# Autodesk Inventor assembly: Rail_assy
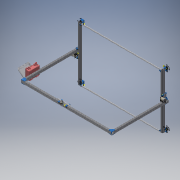
[picture p0: Inventor's stored thumbnail of the model, 180x180]
Saved by Autodesk Inventor 2019.4 (Build 234330000, 330)
## iProperties
Created: 2021-02-01
Part Number: Rail_assy
Document SubType Name: Assembly
Designer: Jorian Brusind
Author: Jorian Brusind
## Documents named in this file (12)
- C:\Users\Jorian Brusind\Documents\GitHub\PersonalProjects\HyperRail\Inventor Files\Rail_assy.iam
- C:\Users\Jorian Brusind\Documents\GitHub\PersonalProjects\HyperRail\Inventor Files\Rail_Assembly.iam
- C:\Users\Jorian Brusind\Documents\GitHub\PersonalProjects\Inventor Projects\Useful models\8020_Sets\IPT_40_Series\Extra_40_Series\HFS5-4060-4000\HFS5-4060-2125.ipt
- C:\Users\Jorian Brusind\Documents\GitHub\PersonalProjects\HyperRail\Inventor Files\YAxis_Carriage.iam
- C:\Users\Jorian Brusind\Documents\GitHub\PersonalProjects\HyperRail\Inventor Files\Small_belt_5mm_1mm.ipt
- C:\Users\Jorian Brusind\Documents\GitHub\PersonalProjects\HyperRail\Inventor Files\90deg_4040Bracket.ipt
- C:\Users\Jorian Brusind\Documents\GitHub\PersonalProjects\Inventor Projects\Useful models\8020_Sets\IPT_20_Series\Extra_20_Series\8020_14057m\14057_m.ipt
- C:\Users\Jorian Brusind\Documents\GitHub\PersonalProjects\HyperRail\Inventor Files\Small_Belt_Clamp.ipt
- C:\Users\Jorian Brusind\Documents\GitHub\PersonalProjects\HyperRail\Inventor Files\Ebox_assy.iam
- C:\Users\Jorian Brusind\Documents\GitHub\PersonalProjects\Inventor Projects\Useful models\8020_Sets\IPT_20_Series\IPT_20_Series\20-2020_1895mm.ipt
- C:\Users\Jorian Brusind\Documents\GitHub\PersonalProjects\HyperRail\Inventor Files\RightAngle_Bracket.ipt
- C:\Users\Jorian Brusind\Documents\GitHub\PersonalProjects\Inventor Projects\Useful models\8020_Sets\IPT_40_Series\Extra_40_Series\90deg_4040.ipt
## Components (23 placed, 11 different names)
1. Rail_Assembly:1 [sub-assembly] — Mate:1, Flush:1, Flush:2, Mate:4, Mate:6, Mate:7, Flush:5, Flush:6, Mate:25, Flush:15, Flush:17, Mate:36, Mate:38, Flush:30, Mate:44
2. HFS5-4060-2125:1 — Mate:1, Flush:1, Flush:2, Mate:5, Flush:3, Flush:4, Mate:8, Mate:9, Mate:10, Mate:12, Mate:13, Mate:14, Flush:8, Flush:10, Mate:20, Flush:11, Flush:14, Mate:24, Mate:26, Flush:16, Mate:27, Flush:18, Mate:28, Flush:19, Flush:20, Mate:29, Flush:21, Flush:22, Mate:31, Mate:43, Flush:32, Mate:45, Flush:33
3. YAxis_Carriage:1 [sub-assembly] — Mate:8, Mate:9, Mate:11, Mate:15
4. Rail_Assembly:2 [sub-assembly] — Mate:5, Flush:3, Flush:4, Flush:6, Mate:16, Flush:7, Mate:17, Flush:9, Mate:19, Mate:30, Flush:23, Mate:32, Flush:24, Flush:25, Mate:33, Flush:26, Flush:27, Mate:35, Flush:28, Mate:41, Flush:31, Mate:42
5. Small_belt_5mm_1mm:1 — Mate:10, Mate:11, Mate:12
6. Small_belt_5mm_1mm:2 — Mate:13, Mate:14, Mate:15
7. 90deg_4040Bracket:1 — Mate:16, Flush:7, Flush:8
8. 90deg_4040Bracket:2 — Mate:17, Flush:9, Flush:10
9. 14057_m:1 — Mate:19, Mate:20, Flush:11
10. 14057_m:4 — Flush:14, Mate:24, Mate:25
11. 90deg_4040Bracket:3 — Mate:26, Flush:15, Flush:16
12. 90deg_4040Bracket:4 — Mate:27, Flush:17, Flush:18
13. Small_Belt_Clamp:1 — Mate:28, Flush:19, Flush:20
14. Small_Belt_Clamp:2 — Mate:29, Flush:21, Flush:22
15. Ebox_assy:1 [sub-assembly] — Mate:30, Flush:23, Mate:31
16. 20-2020_1895mm:1 — Mate:33, Flush:26, Flush:27, Mate:34, Mate:37, Flush:29
17. 20-2020_1895mm:2 — Mate:32, Flush:24, Flush:25, Mate:39, Mate:40
18. RightAngle_Bracket:1 — Mate:34, Mate:35, Flush:28
19. RightAngle_Bracket:2 — Mate:40, Mate:41, Flush:31
20. RightAngle_Bracket:3 — Mate:36, Mate:37, Flush:29
21. RightAngle_Bracket:4 — Mate:38, Mate:39, Flush:30
22. 90deg_4040:1 — Mate:42, Mate:43, Flush:32
23. 90deg_4040:2 — Mate:44, Mate:45, Flush:33
## Relationships (70: Mate 39, Flush 31)
- Mate:1: Rail_Assembly:1 ↔ HFS5-4060-2125:1
- Flush:1: Rail_Assembly:1 ↔ HFS5-4060-2125:1
- Flush:2: Rail_Assembly:1 ↔ HFS5-4060-2125:1
- Mate:4: Rail_Assembly:1
- Mate:5: HFS5-4060-2125:1 ↔ Rail_Assembly:2
- Flush:3: HFS5-4060-2125:1 ↔ Rail_Assembly:2
- Flush:4: HFS5-4060-2125:1 ↔ Rail_Assembly:2
- Mate:6: Rail_Assembly:1
- Mate:7: Rail_Assembly:1
- Flush:5: Rail_Assembly:1
- Flush:6: Rail_Assembly:1 ↔ Rail_Assembly:2
- Mate:8 (7 mm): HFS5-4060-2125:1 ↔ YAxis_Carriage:1
- Mate:9 (-1 mm): HFS5-4060-2125:1 ↔ YAxis_Carriage:1
- Mate:10: HFS5-4060-2125:1 ↔ Small_belt_5mm_1mm:1
- Mate:11: YAxis_Carriage:1 ↔ Small_belt_5mm_1mm:1
- Mate:12 (3.5 mm): HFS5-4060-2125:1 ↔ Small_belt_5mm_1mm:1
- Mate:13: HFS5-4060-2125:1 ↔ Small_belt_5mm_1mm:2
- Mate:14 (0.5 mm): HFS5-4060-2125:1 ↔ Small_belt_5mm_1mm:2
- Mate:15: YAxis_Carriage:1 ↔ Small_belt_5mm_1mm:2
- Mate:16: Rail_Assembly:2 ↔ 90deg_4040Bracket:1
- Flush:7: Rail_Assembly:2 ↔ 90deg_4040Bracket:1
- Flush:8: HFS5-4060-2125:1 ↔ 90deg_4040Bracket:1
- Mate:17: Rail_Assembly:2 ↔ 90deg_4040Bracket:2
- Flush:9: Rail_Assembly:2 ↔ 90deg_4040Bracket:2
- Flush:10: HFS5-4060-2125:1 ↔ 90deg_4040Bracket:2
- Mate:19: Rail_Assembly:2 ↔ 14057_m:1
- Mate:20: HFS5-4060-2125:1 ↔ 14057_m:1
- Flush:11: HFS5-4060-2125:1 ↔ 14057_m:1
- Flush:14: HFS5-4060-2125:1 ↔ 14057_m:4
- Mate:24: HFS5-4060-2125:1 ↔ 14057_m:4
- Mate:25: Rail_Assembly:1 ↔ 14057_m:4
- Mate:26: HFS5-4060-2125:1 ↔ 90deg_4040Bracket:3
- Flush:15: Rail_Assembly:1 ↔ 90deg_4040Bracket:3
- Flush:16: HFS5-4060-2125:1 ↔ 90deg_4040Bracket:3
- Mate:27: HFS5-4060-2125:1 ↔ 90deg_4040Bracket:4
- Flush:17: Rail_Assembly:1 ↔ 90deg_4040Bracket:4
- Flush:18: HFS5-4060-2125:1 ↔ 90deg_4040Bracket:4
- Mate:28: HFS5-4060-2125:1 ↔ Small_Belt_Clamp:1
- Flush:19: HFS5-4060-2125:1 ↔ Small_Belt_Clamp:1
- Flush:20: HFS5-4060-2125:1 ↔ Small_Belt_Clamp:1
- Mate:29: HFS5-4060-2125:1 ↔ Small_Belt_Clamp:2
- Flush:21: HFS5-4060-2125:1 ↔ Small_Belt_Clamp:2
- Flush:22: HFS5-4060-2125:1 ↔ Small_Belt_Clamp:2
- Mate:30: Rail_Assembly:2 ↔ Ebox_assy:1
- Flush:23: Rail_Assembly:2 ↔ Ebox_assy:1
- Mate:31 (-200 mm): HFS5-4060-2125:1 ↔ Ebox_assy:1
- Mate:32: Rail_Assembly:2 ↔ 20-2020_1895mm:2
- Flush:24: Rail_Assembly:2 ↔ 20-2020_1895mm:2
- Flush:25: Rail_Assembly:2 ↔ 20-2020_1895mm:2
- Mate:33: Rail_Assembly:2 ↔ 20-2020_1895mm:1
- Flush:26: Rail_Assembly:2 ↔ 20-2020_1895mm:1
- Flush:27: Rail_Assembly:2 ↔ 20-2020_1895mm:1
- Mate:34: 20-2020_1895mm:1 ↔ RightAngle_Bracket:1
- Mate:35: Rail_Assembly:2 ↔ RightAngle_Bracket:1
- Flush:28 (-3 mm): Rail_Assembly:2 ↔ RightAngle_Bracket:1
- Mate:36: Rail_Assembly:1 ↔ RightAngle_Bracket:3
- Mate:37: 20-2020_1895mm:1 ↔ RightAngle_Bracket:3
- Flush:29 (-3 mm): 20-2020_1895mm:1 ↔ RightAngle_Bracket:3
- Mate:38: Rail_Assembly:1 ↔ RightAngle_Bracket:4
- Mate:39: 20-2020_1895mm:2 ↔ RightAngle_Bracket:4
- Flush:30 (3 mm): Rail_Assembly:1 ↔ RightAngle_Bracket:4
- Mate:40: 20-2020_1895mm:2 ↔ RightAngle_Bracket:2
- Mate:41: Rail_Assembly:2 ↔ RightAngle_Bracket:2
- Flush:31 (-3 mm): Rail_Assembly:2 ↔ RightAngle_Bracket:2
- Mate:42: Rail_Assembly:2 ↔ 90deg_4040:1
- Mate:43: HFS5-4060-2125:1 ↔ 90deg_4040:1
- Flush:32: HFS5-4060-2125:1 ↔ 90deg_4040:1
- Mate:44: Rail_Assembly:1 ↔ 90deg_4040:2
- Mate:45: HFS5-4060-2125:1 ↔ 90deg_4040:2
- Flush:33: HFS5-4060-2125:1 ↔ 90deg_4040:2
